# Autodesk Inventor assembly: ensamble
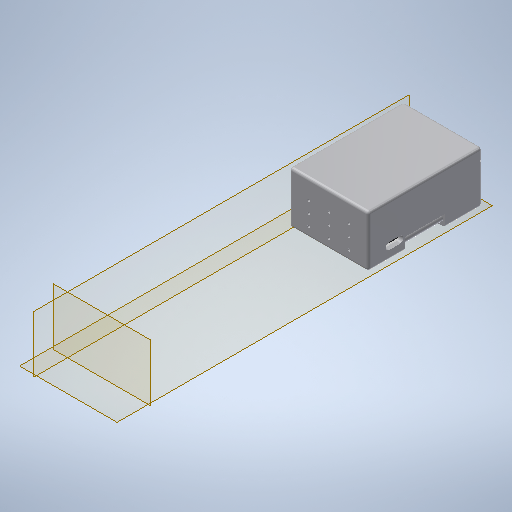
[picture p0: Inventor's stored thumbnail of the model, 512x512]
Saved by Autodesk Inventor 2025.2 (Build 292293000, 293)
## iProperties
Created: 2025-10-17
Part Number: ensamble
Material: Generic
Document SubType Name: Assembly
Designer: Ricardo
Author: Ricardo
## Documents named in this file (8)
- C:\Users\Ricardo\Documents\Inventor\TFC\ensamble.iam
- C:\Users\Ricardo\Documents\Inventor\TFC\Componentes\d-sun-dc-dc-step-down-voltage-regulator-simple-version-1.snapshot.4\PCB COMPLETA.iam
- C:\Users\Ricardo\Documents\Inventor\TFC\Base.ipt
- C:\Users\Ricardo\Documents\Inventor\TFC\Componentes\motor.ipt
- C:\Users\Ricardo\Documents\Inventor\TFC\Componentes\esp32_devkitv1-1.snapshot.7\ESP32_DevKitV1\ESP32_DevKitV1_en.ipt
- C:\Users\Ricardo\Documents\Inventor\TFC\superior.ipt
- C:\Users\Ricardo\Documents\Inventor\TFC\Componentes\push-switch-8x8-6pin-with-lock-1.snapshot.1\LatchSwitch_7x7\LatchSwitch_7x7\LatchSwitch_7x7_ens.ipt
- C:\Users\Ricardo\Documents\Inventor\Content Center Files\R2025\en-US\ISO 4017(1)\ISO 4017 - M2 x 4 - ISO.ipt
## Components (10 placed, 7 different names)
1. PCB COMPLETA:1 [sub-assembly] — Mate:9, Mate:10, Mate:11, Mate:15, Mate:16, Mate:17, Mate:22, Mate:24, Mate:26, Mate:28
2. Base:1 — Mate:3, Mate:9, Mate:10, Mate:11, Flush:1, Flush:2, Mate:12, Mate:13, Mate:14, Mate:18, Insert:5, Mate:19, Mate:20, Mate:21, Mate:23, Mate:25, Mate:27
3. motor:1 — Mate:3, Insert:5
4. ESP32_DevKitV1_en:1 — Mate:15, Mate:16, Mate:17
5. superior:1 — Flush:1, Flush:2, Mate:18
6. LatchSwitch_7x7_ens:1 — Mate:12, Mate:13, Mate:14
7. ISO 4017 M2 x 4:1 — Mate:21, Mate:22
8. ISO 4017 M2 x 4:2 — Mate:23, Mate:24
9. ISO 4017 M2 x 4:3 — Mate:25, Mate:26
10. ISO 4017 M2 x 4:4 — Mate:27, Mate:28
## Relationships (24: Mate 21, Flush 2, Insert 1)
- Mate:3: Base:1 ↔ motor:1
- Mate:9 (1 mm): PCB COMPLETA:1 ↔ Base:1
- Mate:10 (0.5 mm): PCB COMPLETA:1 ↔ Base:1
- Mate:11: PCB COMPLETA:1 ↔ Base:1
- Flush:1: Base:1 ↔ superior:1
- Flush:2: Base:1 ↔ superior:1
- Mate:12 (-6.5 mm): Base:1 ↔ LatchSwitch_7x7_ens:1
- Mate:13: Base:1 ↔ LatchSwitch_7x7_ens:1
- Mate:14: Base:1 ↔ LatchSwitch_7x7_ens:1
- Mate:15: PCB COMPLETA:1 ↔ ESP32_DevKitV1_en:1
- Mate:16: PCB COMPLETA:1 ↔ ESP32_DevKitV1_en:1
- Mate:17: PCB COMPLETA:1 ↔ ESP32_DevKitV1_en:1
- Mate:18: Base:1 ↔ superior:1
- Insert:5: Base:1 ↔ motor:1
- Mate:19: Base:1
- Mate:20: Base:1
- Mate:21: Base:1 ↔ ISO 4017 M2 x 4:1
- Mate:22: PCB COMPLETA:1 ↔ ISO 4017 M2 x 4:1
- Mate:23: Base:1 ↔ ISO 4017 M2 x 4:2
- Mate:24: PCB COMPLETA:1 ↔ ISO 4017 M2 x 4:2
- Mate:25: Base:1 ↔ ISO 4017 M2 x 4:3
- Mate:26: PCB COMPLETA:1 ↔ ISO 4017 M2 x 4:3
- Mate:27: Base:1 ↔ ISO 4017 M2 x 4:4
- Mate:28: PCB COMPLETA:1 ↔ ISO 4017 M2 x 4:4
